# Autodesk Inventor assembly: standoff_brace_front
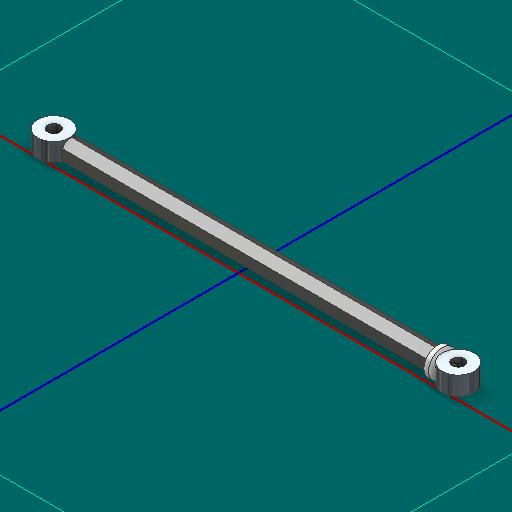
[picture p0: Inventor's stored thumbnail of the model, 512x512]
Saved by Autodesk Inventor 2025 (Build 290162000, 162)
## iProperties
Created: 2024-08-17
Part Number: standoff_brace_front
Document SubType Name: Assembly
Designer: averey
Author: averey
## Documents named in this file (6)
- C:\Users\avere\vex_robotics_high_stakes\hardware\cad\ATLAS\chassis\structure\standoff_brace_front.iam
- C:\Users\avere\vex_robotics_high_stakes\hardware\cad\VEX-CAD-Inventor\Motion\Shaft LS\Shaft Collar ipts\Shaft Collar No Screw.ipt
- C:\Users\avere\vex_robotics_high_stakes\hardware\cad\VEX-CAD-Inventor\Structure\Standoff\Standoff 5.00.ipt
- C:\Users\avere\vex_robotics_high_stakes\hardware\cad\VEX-CAD-Inventor\Structure\Standoff.ipt
- C:\Users\avere\vex_robotics_high_stakes\hardware\cad\VEX-CAD-Inventor\Motion\Spacers\Washer Teflon\TWasher .375 OD x .06250.ipt
- C:\Users\avere\vex_robotics_high_stakes\hardware\cad\VEX-CAD-Inventor\Motion\Spacers\Washer Teflon.ipt
## Components (4 placed, 3 different names)
1. Shaft Collar No Screw:1 — Angle:2
2. Shaft Collar No Screw:2 — Angle:1
3. Standoff 5.00:1
4. TWasher .375 OD x .06250:1
## Relationships (6: Insert 3, Angle 2, Mate 1)
- [Mate]: Shaft Collar No Screw:1 ↔ Shaft Collar No Screw:2
- [Insert]: Standoff 5.00:1 ↔ TWasher .375 OD x .06250:1
- [Insert]: Shaft Collar No Screw:2 ↔ TWasher .375 OD x .06250:1
- [Insert] (128.7 mm): Shaft Collar No Screw:1 ↔ Shaft Collar No Screw:2
- Angle:1 (0 deg): Shaft Collar No Screw:2
- Angle:2 (0 deg): Shaft Collar No Screw:1
